# Autodesk Inventor assembly: Motor_Tire_Assy
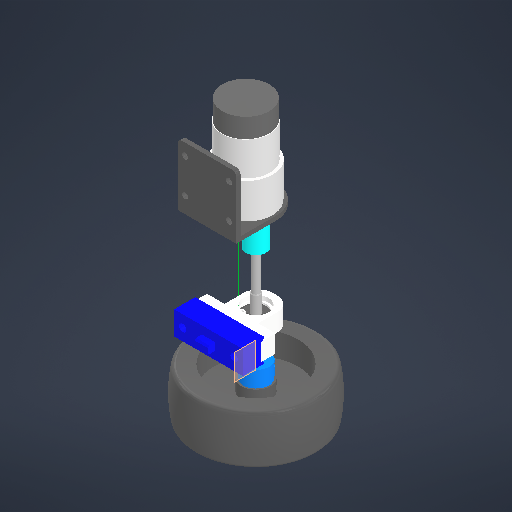
[picture p0: Inventor's stored thumbnail of the model, 512x512]
Saved by Autodesk Inventor 2026.2 (Build 302298010, 298A)
## iProperties
Created: 2026-06-01
Part Number: Motor_Tire_Assy
Document SubType Name: Assembly
Designer: dalbi
Author: dalbi
## Documents named in this file (7)
- C:\Users\User\Desktop\트리보 관련 자료\최종 설계 파일(조립시 참고할 파일)\Motor_Tire_Assy.iam
- C:\Users\User\Desktop\트리보 관련 자료\최종 설계 파일(조립시 참고할 파일)\VPK 설계파일(최종본 아님)\P_BEARING_C-BGHPA606ZZ-20.ipt
- C:\Users\User\Desktop\트리보 관련 자료\최종 설계 파일(조립시 참고할 파일)\VPK 설계파일(최종본 아님)\P_MOTOR_FIXED_BRACKET.ipt
- C:\Users\User\Desktop\트리보 관련 자료\최종 설계 파일(조립시 참고할 파일)\VPK 설계파일(최종본 아님)\P_MOTOR_GM37-520 12V 1_90.ipt
- C:\Users\User\Desktop\트리보 관련 자료\최종 설계 파일(조립시 참고할 파일)\VPK 설계파일(최종본 아님)\P_Tire_85mm Block Rubber.ipt
- C:\Users\User\Desktop\트리보 관련 자료\최종 설계 파일(조립시 참고할 파일)\VPK 설계파일(최종본 아님)\P_Shaft D6_with_Coupling.ipt
- C:\Users\User\Desktop\트리보 관련 자료\최종 설계 파일(조립시 참고할 파일)\Bearing Spacer_V2.ipt
## Components (6 placed, 6 different names)
1. P_BEARING_C-BGHPA606ZZ-20.1 — 메이트:5, 메이트:6, 메이트:7, 메이트:8
2. P_MOTOR_FIXED_BRACKET.1 — 메이트:9, 메이트:10
3. P_MOTOR_GM37-520 12V 1_90.1 — 메이트:1, 메이트:4, 메이트:9, 메이트:10
4. P_Tire_85mm Block Rubber.1 — 메이트:2, 메이트:3, 메이트:5
5. P_Shaft D6_with_Coupling.1 — 메이트:1, 메이트:2, 메이트:3, 메이트:4, 메이트:8
6. Bearing Spacer_V2:1 — 메이트:6, 메이트:7
## Relationships (10: Mate 10)
- 메이트:1 [Mate]: P_MOTOR_GM37-520 12V 1_90.1 ↔ P_Shaft D6_with_Coupling.1
- 메이트:2 [Mate]: P_Tire_85mm Block Rubber.1 ↔ P_Shaft D6_with_Coupling.1
- 메이트:3 [Mate]: P_Tire_85mm Block Rubber.1 ↔ P_Shaft D6_with_Coupling.1
- 메이트:4 [Mate]: P_MOTOR_GM37-520 12V 1_90.1 ↔ P_Shaft D6_with_Coupling.1
- 메이트:5 [Mate] (20 mm): P_BEARING_C-BGHPA606ZZ-20.1 ↔ P_Tire_85mm Block Rubber.1
- 메이트:6 [Mate]: P_BEARING_C-BGHPA606ZZ-20.1 ↔ Bearing Spacer_V2:1
- 메이트:7 [Mate]: P_BEARING_C-BGHPA606ZZ-20.1 ↔ Bearing Spacer_V2:1
- 메이트:8 [Mate]: P_BEARING_C-BGHPA606ZZ-20.1 ↔ P_Shaft D6_with_Coupling.1
- 메이트:9 [Mate]: P_MOTOR_FIXED_BRACKET.1 ↔ P_MOTOR_GM37-520 12V 1_90.1
- 메이트:10 [Mate]: P_MOTOR_FIXED_BRACKET.1 ↔ P_MOTOR_GM37-520 12V 1_90.1
